# Autodesk Inventor assembly: Eierkocher
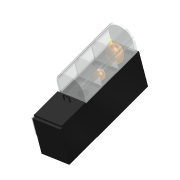
[picture p0: Inventor's stored thumbnail of the model, 180x180]
Saved by Autodesk Inventor 2020 (Build 240168000, 168)
## iProperties
Created: 2022-01-25
Part Number: Eierkocher
Document SubType Name: Assembly
Designer: Julian Uhl
Author: Julian Uhl
## Documents named in this file (12)
- C:\Schule\Eier-Inventor\Eierkocher.iam
- C:\Schule\Eier-Inventor\EierkocherTeil1.ipt
- C:\Schule\Eier-Inventor\EierkocherTeil2.ipt
- C:\Schule\Eier-Inventor\Eihalter.ipt
- C:\Schule\Eier-Inventor\Raspberry_Dummy.ipt
- C:\Schule\Eier-Inventor\Display_Dummy.ipt
- C:\Schule\Eier-Inventor\DeckelMess.ipt
- C:\Schule\Eier-Inventor\Ei_groß.ipt
- C:\Schule\Eier-Inventor\Eihalter_Halter.ipt
- C:\Schule\Eier-Inventor\Ei.ipt
- C:\Schule\Eier-Inventor\DeckelKoch_Better.ipt
- C:\Schule\Eier-Inventor\Dichtung_1.ipt
## Components (24 placed, 11 different names)
1. EierkocherTeil1:1 — Fluchtend:1, Passend:1, Fluchtend:2, Passend:2, Passend:3, Passend:4, Passend:5, Passend:6, Passend:7, Passend:16, Passend:17, Passend:18, Passend:19, Passend:20, Fluchtend:8, Passend:21, Passend:22, Fluchtend:9, Passend:23, Passend:24, Fluchtend:10, Passend:26, Passend:27, Fluchtend:11, Passend:28, Fluchtend:12, Passend:29, Passend:30, Fluchtend:13, Passend:31, Passend:32, Fluchtend:14, Passend:33, Passend:35, Passend:36, Fluchtend:15, Passend:37, Passend:38, Fluchtend:16, Passend:39, Passend:40, Fluchtend:17, Passend:41, Passend:42, Fluchtend:18, Passend:48, Passend:49, Passend:50, Passend:51, Passend:52
2. EierkocherTeil2:1 — Fluchtend:1, Passend:1, Fluchtend:2, Passend:8, Fluchtend:3, Fluchtend:4, Fluchtend:5, Fluchtend:6, Passend:9, Fluchtend:7, Passend:10, Passend:11, Passend:12
3. Eihalter:1 — Passend:2, Passend:3, Passend:25
4. Eihalter:2 — Passend:4, Passend:5, Passend:34, Passend:46
5. Eihalter:3 — Passend:6, Passend:7, Passend:43, Passend:44, Passend:45
6. Raspberry_Dummy:1 — Passend:10, Passend:11, Passend:12
7. Display_Dummy:1 — Passend:8, Fluchtend:3, Fluchtend:4
8. DeckelMess:2 — Fluchtend:5, Fluchtend:6, Passend:9, Fluchtend:7
9. Ei_groß:1 — Passend:44, Passend:45
10. Eihalter_Halter:1 — Passend:19, Passend:20, Fluchtend:8
11. Eihalter_Halter:2 — Passend:21, Passend:22, Fluchtend:9
12. Eihalter_Halter:3 — Passend:23, Passend:24, Fluchtend:10
13. Eihalter_Halter:4 — Passend:16, Passend:17, Passend:18, Passend:25
14. Eihalter_Halter:5 — Passend:26, Passend:27, Fluchtend:11
15. Eihalter_Halter:6 — Passend:28, Fluchtend:12, Passend:29
16. Eihalter_Halter:7 — Passend:32, Fluchtend:14, Passend:33, Passend:34
17. Eihalter_Halter:8 — Passend:30, Fluchtend:13, Passend:31
18. Eihalter_Halter:9 — Passend:35, Passend:36, Fluchtend:15
19. Eihalter_Halter:10 — Passend:39, Passend:40, Fluchtend:17, Passend:43
20. Eihalter_Halter:11 — Passend:41, Passend:42, Fluchtend:18
21. Eihalter_Halter:12 — Passend:37, Passend:38, Fluchtend:16
22. Ei:1 — Passend:46
23. DeckelKoch_Better:1 — Passend:48, Passend:49, Passend:53
24. Dichtung_1:1 — Passend:50, Passend:51, Passend:52, Passend:53
## Relationships (67: Mate 49, Flush 18)
- Fluchtend:1 [Flush]: EierkocherTeil1:1 ↔ EierkocherTeil2:1
- Passend:1 [Mate]: EierkocherTeil1:1 ↔ EierkocherTeil2:1
- Fluchtend:2 [Flush]: EierkocherTeil1:1 ↔ EierkocherTeil2:1
- Passend:2 [Mate]: EierkocherTeil1:1 ↔ Eihalter:1
- Passend:3 [Mate]: EierkocherTeil1:1 ↔ Eihalter:1
- Passend:4 [Mate]: EierkocherTeil1:1 ↔ Eihalter:2
- Passend:5 [Mate]: EierkocherTeil1:1 ↔ Eihalter:2
- Passend:6 [Mate]: EierkocherTeil1:1 ↔ Eihalter:3
- Passend:7 [Mate]: EierkocherTeil1:1 ↔ Eihalter:3
- Passend:8 [Mate]: EierkocherTeil2:1 ↔ Display_Dummy:1
- Fluchtend:3 [Flush] (10 mm): EierkocherTeil2:1 ↔ Display_Dummy:1
- Fluchtend:4 [Flush] (10 mm): EierkocherTeil2:1 ↔ Display_Dummy:1
- Fluchtend:5 [Flush]: EierkocherTeil2:1 ↔ DeckelMess:2
- Fluchtend:6 [Flush]: EierkocherTeil2:1 ↔ DeckelMess:2
- Passend:9 [Mate]: EierkocherTeil2:1 ↔ DeckelMess:2
- Fluchtend:7 [Flush]: EierkocherTeil2:1 ↔ DeckelMess:2
- Passend:10 [Mate]: EierkocherTeil2:1 ↔ Raspberry_Dummy:1
- Passend:11 [Mate] (20 mm): EierkocherTeil2:1 ↔ Raspberry_Dummy:1
- Passend:12 [Mate] (15 mm): EierkocherTeil2:1 ↔ Raspberry_Dummy:1
- Passend:16 [Mate]: EierkocherTeil1:1 ↔ Eihalter_Halter:4
- Passend:17 [Mate]: EierkocherTeil1:1 ↔ Eihalter_Halter:4
- Passend:18 [Mate] (-25 mm): EierkocherTeil1:1 ↔ Eihalter_Halter:4
- Passend:19 [Mate]: EierkocherTeil1:1 ↔ Eihalter_Halter:1
- Passend:20 [Mate]: EierkocherTeil1:1 ↔ Eihalter_Halter:1
- Fluchtend:8 [Flush] (25 mm): EierkocherTeil1:1 ↔ Eihalter_Halter:1
- Passend:21 [Mate]: EierkocherTeil1:1 ↔ Eihalter_Halter:2
- Passend:22 [Mate]: EierkocherTeil1:1 ↔ Eihalter_Halter:2
- Fluchtend:9 [Flush] (25 mm): EierkocherTeil1:1 ↔ Eihalter_Halter:2
- Passend:23 [Mate]: EierkocherTeil1:1 ↔ Eihalter_Halter:3
- Passend:24 [Mate]: EierkocherTeil1:1 ↔ Eihalter_Halter:3
- Fluchtend:10 [Flush] (25 mm): EierkocherTeil1:1 ↔ Eihalter_Halter:3
- Passend:25 [Mate]: Eihalter:1 ↔ Eihalter_Halter:4
- Passend:26 [Mate]: EierkocherTeil1:1 ↔ Eihalter_Halter:5
- Passend:27 [Mate]: EierkocherTeil1:1 ↔ Eihalter_Halter:5
- Fluchtend:11 [Flush] (25 mm): EierkocherTeil1:1 ↔ Eihalter_Halter:5
- Passend:28 [Mate]: EierkocherTeil1:1 ↔ Eihalter_Halter:6
- Fluchtend:12 [Flush] (25 mm): EierkocherTeil1:1 ↔ Eihalter_Halter:6
- Passend:29 [Mate]: EierkocherTeil1:1 ↔ Eihalter_Halter:6
- Passend:30 [Mate]: EierkocherTeil1:1 ↔ Eihalter_Halter:8
- Fluchtend:13 [Flush] (25 mm): EierkocherTeil1:1 ↔ Eihalter_Halter:8
- Passend:31 [Mate]: EierkocherTeil1:1 ↔ Eihalter_Halter:8
- Passend:32 [Mate]: EierkocherTeil1:1 ↔ Eihalter_Halter:7
- Fluchtend:14 [Flush] (25 mm): EierkocherTeil1:1 ↔ Eihalter_Halter:7
- Passend:33 [Mate]: EierkocherTeil1:1 ↔ Eihalter_Halter:7
- Passend:34 [Mate]: Eihalter:2 ↔ Eihalter_Halter:7
- Passend:35 [Mate]: EierkocherTeil1:1 ↔ Eihalter_Halter:9
- Passend:36 [Mate]: EierkocherTeil1:1 ↔ Eihalter_Halter:9
- Fluchtend:15 [Flush] (25 mm): EierkocherTeil1:1 ↔ Eihalter_Halter:9
- Passend:37 [Mate]: EierkocherTeil1:1 ↔ Eihalter_Halter:12
- Passend:38 [Mate]: EierkocherTeil1:1 ↔ Eihalter_Halter:12
- Fluchtend:16 [Flush] (25 mm): EierkocherTeil1:1 ↔ Eihalter_Halter:12
- Passend:39 [Mate]: EierkocherTeil1:1 ↔ Eihalter_Halter:10
- Passend:40 [Mate]: EierkocherTeil1:1 ↔ Eihalter_Halter:10
- Fluchtend:17 [Flush] (25 mm): EierkocherTeil1:1 ↔ Eihalter_Halter:10
- Passend:41 [Mate]: EierkocherTeil1:1 ↔ Eihalter_Halter:11
- Passend:42 [Mate]: EierkocherTeil1:1 ↔ Eihalter_Halter:11
- Fluchtend:18 [Flush] (25 mm): EierkocherTeil1:1 ↔ Eihalter_Halter:11
- Passend:43 [Mate]: Eihalter:3 ↔ Eihalter_Halter:10
- Passend:44 [Mate]: Eihalter:3 ↔ Ei_groß:1
- Passend:45 [Mate] (30 mm): Eihalter:3 ↔ Ei_groß:1
- Passend:46 [Mate] (1 mm): Eihalter:2 ↔ Ei:1
- Passend:48 [Mate]: EierkocherTeil1:1 ↔ DeckelKoch_Better:1
- Passend:49 [Mate]: EierkocherTeil1:1 ↔ DeckelKoch_Better:1
- Passend:50 [Mate]: EierkocherTeil1:1 ↔ Dichtung_1:1
- Passend:51 [Mate] (1 mm): EierkocherTeil1:1 ↔ Dichtung_1:1
- Passend:52 [Mate] (1 mm): EierkocherTeil1:1 ↔ Dichtung_1:1
- Passend:53 [Mate]: DeckelKoch_Better:1 ↔ Dichtung_1:1
